# Autodesk Inventor assembly: Encoder
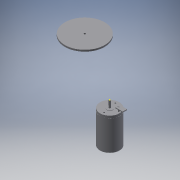
[picture p0: Inventor's stored thumbnail of the model, 180x180]
Saved by Autodesk Inventor 2016 (Build 200138000, 138)
## iProperties
Created: 2016-11-30
Part Number: Encoder
Document SubType Name: Assembly
Designer: Student
Author: Student
## Documents named in this file (5)
- C:\Users\Student\Desktop\Noah Code\Encoder.iam
- C:\Users\Student\Documents\motor MABCHI 3W Noah.ipt
- C:\Users\Student\Documents\Encoder wheel Noah.ipt
- C:\Users\Student\Documents\encoder noah.ipt
- C:\Users\Student\Documents\encoder mount noah.ipt
## Components (4 placed, 4 different names)
1. motor MABCHI 3W Noah:1 — Rotational:1
2. encoder noah:1 — Mate:1
3. Encoder wheel Noah:1
4. encoder mount noah:1 — Rotational:1, Mate:1
## Relationships (2: RevoluteJoint 1, Mate 1)
- Rotational:1 [RevoluteJoint]: motor MABCHI 3W Noah:1 ↔ encoder mount noah:1
- Mate:1: encoder noah:1 ↔ encoder mount noah:1
